# Autodesk Inventor assembly: FullAssembly
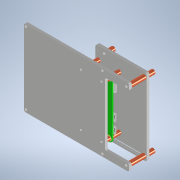
[picture p0: Inventor's stored thumbnail of the model, 180x180]
Saved by Autodesk Inventor 2021.1 (Build 251245010, 245A)
## iProperties
Created: 2025-08-17
Part Number: FullAssembly
Document SubType Name: Assembly
Designer: TUAN PC
Author: TUAN PC
## Documents named in this file (8)
- H:\01_GitProject\99_Learning\06_RPi0_Case\FullAssembly.iam
- H:\01_GitProject\99_Learning\06_RPi0_Case\00_BottomPart.ipt
- H:\01_GitProject\99_Learning\06_RPi0_Case\03_Column25_short.ipt
- H:\01_GitProject\99_Learning\06_RPi0_Case\Raspberry Pi Zero 2 W.ipt
- H:\01_GitProject\99_Learning\06_RPi0_Case\02_Column25_long.ipt
- H:\01_GitProject\99_Learning\06_RPi0_Case\01_TopPart.ipt
- H:\01_GitProject\99_Learning\06_RPi0_Case\04_Column30_short.ipt
- H:\01_GitProject\99_Learning\06_RPi0_Case\05_Column30_long.ipt
## Components (17 placed, 7 different names)
1. 00_BottomPart:1 — Mate:1, Mate:2, Mate:3, Mate:4, Mate:5, Mate:6, Mate:7, Mate:8, Mate:31, Mate:32, Mate:33, Mate:34
2. 03_Column25_short:1 — Mate:2, Mate:7
3. 03_Column25_short:2 — Mate:1, Mate:6, Mate:11
4. 03_Column25_short:3 — Mate:3, Mate:8, Mate:10
5. 03_Column25_short:4 — Mate:4, Mate:5, Mate:9
6. Raspberry Pi Zero 2 W:1 — Mate:9, Mate:10, Mate:11, Mate:12, Mate:13, Mate:14, Mate:15, Mate:16, Mate:17, Mate:18, Mate:19
7. 02_Column25_long:1 — Mate:13, Mate:18, Mate:20, Mate:21
8. 02_Column25_long:2 — Mate:12, Mate:19
9. 02_Column25_long:3 — Mate:15, Mate:16, Mate:22
10. 02_Column25_long:4 — Mate:14, Mate:17
11. 01_TopPart:1 — Mate:20, Mate:21, Mate:22, Mate:23, Mate:24, Mate:25, Mate:26, Mate:27, Mate:28, Mate:29, Mate:30
12. 04_Column30_short:1 — Mate:23, Mate:28
13. 04_Column30_short:2 — Mate:24, Mate:29
14. 04_Column30_short:3 — Mate:25, Mate:30
15. 04_Column30_short:4 — Mate:26, Mate:27
16. 05_Column30_long:1 — Mate:32, Mate:34
17. 05_Column30_long:2 — Mate:31, Mate:33
## Relationships (34: Mate 34)
- Mate:1: 00_BottomPart:1 ↔ 03_Column25_short:2
- Mate:2: 00_BottomPart:1 ↔ 03_Column25_short:1
- Mate:3: 00_BottomPart:1 ↔ 03_Column25_short:3
- Mate:4: 00_BottomPart:1 ↔ 03_Column25_short:4
- Mate:5: 00_BottomPart:1 ↔ 03_Column25_short:4
- Mate:6: 00_BottomPart:1 ↔ 03_Column25_short:2
- Mate:7: 00_BottomPart:1 ↔ 03_Column25_short:1
- Mate:8: 00_BottomPart:1 ↔ 03_Column25_short:3
- Mate:9: 03_Column25_short:4 ↔ Raspberry Pi Zero 2 W:1
- Mate:10: 03_Column25_short:3 ↔ Raspberry Pi Zero 2 W:1
- Mate:11: 03_Column25_short:2 ↔ Raspberry Pi Zero 2 W:1
- Mate:12: Raspberry Pi Zero 2 W:1 ↔ 02_Column25_long:2
- Mate:13: Raspberry Pi Zero 2 W:1 ↔ 02_Column25_long:1
- Mate:14: Raspberry Pi Zero 2 W:1 ↔ 02_Column25_long:4
- Mate:15: Raspberry Pi Zero 2 W:1 ↔ 02_Column25_long:3
- Mate:16: Raspberry Pi Zero 2 W:1 ↔ 02_Column25_long:3
- Mate:17: Raspberry Pi Zero 2 W:1 ↔ 02_Column25_long:4
- Mate:18: Raspberry Pi Zero 2 W:1 ↔ 02_Column25_long:1
- Mate:19: Raspberry Pi Zero 2 W:1 ↔ 02_Column25_long:2
- Mate:20: 02_Column25_long:1 ↔ 01_TopPart:1
- Mate:21: 02_Column25_long:1 ↔ 01_TopPart:1
- Mate:22: 02_Column25_long:3 ↔ 01_TopPart:1
- Mate:23: 01_TopPart:1 ↔ 04_Column30_short:1
- Mate:24: 01_TopPart:1 ↔ 04_Column30_short:2
- Mate:25: 01_TopPart:1 ↔ 04_Column30_short:3
- Mate:26: 01_TopPart:1 ↔ 04_Column30_short:4
- Mate:27: 01_TopPart:1 ↔ 04_Column30_short:4
- Mate:28: 01_TopPart:1 ↔ 04_Column30_short:1
- Mate:29: 01_TopPart:1 ↔ 04_Column30_short:2
- Mate:30: 01_TopPart:1 ↔ 04_Column30_short:3
- Mate:31: 00_BottomPart:1 ↔ 05_Column30_long:2
- Mate:32: 00_BottomPart:1 ↔ 05_Column30_long:1
- Mate:33: 00_BottomPart:1 ↔ 05_Column30_long:2
- Mate:34: 00_BottomPart:1 ↔ 05_Column30_long:1
